# Autodesk Inventor assembly: Eje z base
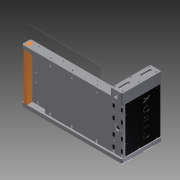
[picture p0: Inventor's stored thumbnail of the model, 180x180]
Saved by Autodesk Inventor 2012 SP1 (Build 160190100, 190)
## iProperties
Created: 2014-12-27
Part Number: Eje z base
Document SubType Name: Assembly
Designer: PRINCIPAL
Author: PRINCIPAL
## Documents named in this file (13)
- E:\impresora juan marc albert\Ultima modificacio Impresora\modificacio chasis 1-9-14\eje z nuevo\Eje z base.iam
- E:\impresora juan marc albert\Ultima modificacio Impresora\modificacio chasis 1-9-14\eje z nuevo\brazo eje z.ipt
- E:\impresora juan marc albert\cojinete lm10uu.ipt
- E:\impresora juan marc albert\Ultima modificacio Impresora\modificacio chasis 1-9-14\eje z nuevo\pieza central base superior.ipt
- E:\impresora juan marc albert\Ultima modificacio Impresora\modificacio chasis 1-9-14\eje z nuevo\pieza central base inferior.ipt
- E:\impresora juan marc albert\Ultima modificacio Impresora\modificacio chasis 1-9-14\eje z nuevo\frontal mes nom.ipt
- E:\impresora juan marc albert\Ultima modificacio Impresora\modificacio chasis 1-9-14\eje z nuevo\base.ipt
- E:\impresora juan marc albert\Ultima modificacio Impresora\modificacio chasis 1-9-14\eje z nuevo\IMAN + ESFERA 6.ipt
- E:\impresora juan marc albert\Ultima modificacio Impresora\modificacio chasis 1-9-14\eje z nuevo\suport iman.ipt
- E:\impresora juan marc albert\Ultima modificacio Impresora\modificacio chasis 1-9-14\eje z nuevo\suport z darrera.ipt
- E:\impresora juan marc albert\Ultima modificacio Impresora\modificacio chasis 1-9-14\eje z nuevo\frontal base reforç.ipt
- E:\impresora juan marc albert\Ultima modificacio Impresora\modificacio chasis 1-9-14\eje z nuevo\suplemento cojinete.ipt
- E:\impresora juan marc albert\Ultima modificacio Impresora\modificacio chasis 1-9-14\eje z nuevo\suplemento cojinete tapa.ipt
## Components (22 placed, 12 different names)
1. brazo eje z:1 — Coincidencia:1, Coincidencia:2, Tangente:1, Tangente:2, Tangente:3, Tangente:4, Ángulo:1, Ángulo:2, Nivelación:1, Nivelación:2, Nivelación:5, Coincidencia:6, Nivelación:4, Coincidencia:14
2. brazo eje z:2 — Coincidencia:3, Coincidencia:4, Tangente:5, Tangente:6, Tangente:7, Tangente:8, Tangente:9, Ángulo:1, Ángulo:2, Nivelación:1, Nivelación:2, Nivelación:3, Coincidencia:5, Nivelación:6, Coincidencia:11, Coincidencia:12, Nivelación:10, Coincidencia:17, Insertar:29
3. cojinete lm10uu:1 — Coincidencia:4, Tangente:8, Tangente:9
4. cojinete lm10uu:2 — Coincidencia:3, Tangente:5, Tangente:6, Tangente:7
5. cojinete lm10uu:3 — Coincidencia:2, Tangente:1, Tangente:2
6. cojinete lm10uu:4 — Coincidencia:1, Tangente:3, Tangente:4
7. pieza central base superior:1 — Nivelación:3, Coincidencia:5, Nivelación:4, Nivelación:5, Ángulo:3, Ángulo:5, Ángulo:6, Ángulo:7, Insertar:17, Insertar:18, Insertar:19, Insertar:20, Insertar:21, Insertar:22
8. pieza central base inferior:1 — Coincidencia:6, Nivelación:6, Nivelación:11, Coincidencia:15, Coincidencia:16
9. frontal mes nom:1 — Coincidencia:11, Coincidencia:12, Nivelación:10, Ángulo:4
10. base:1 — Ángulo:3, Ángulo:4, Insertar:26, Insertar:27, Insertar:28
11. IMAN + ESFERA 6:1 — Insertar:25, Insertar:28
12. IMAN + ESFERA 6:2 — Insertar:24, Insertar:26
13. IMAN + ESFERA 6:3 — Insertar:23, Insertar:27
14. suport iman:1 — Ángulo:6, Insertar:17, Insertar:18, Insertar:23
15. suport iman:2 — Ángulo:7, Insertar:19, Insertar:20, Insertar:24
16. suport iman:3 — Ángulo:5, Insertar:21, Insertar:22, Insertar:25
17. suport z darrera:1 — Nivelación:11, Coincidencia:14
18. frontal base reforç:1 — Coincidencia:15, Coincidencia:16, Coincidencia:17
19. suplemento cojinete:1 — Insertar:29, Insertar:30, Insertar:31
20. suplemento cojinete tapa:1 — Insertar:34
21. suplemento cojinete:2 — Insertar:30, Insertar:31, Insertar:32, Insertar:33
22. suplemento cojinete:3 — Insertar:32, Insertar:33, Insertar:34
## Relationships (54: Insert 18, Mate 12, Tangent 9, Flush 8, Angle 7)
- Coincidencia:1 [Mate]: brazo eje z:1 ↔ cojinete lm10uu:4
- Coincidencia:2 [Mate]: brazo eje z:1 ↔ cojinete lm10uu:3
- Coincidencia:3 [Mate]: brazo eje z:2 ↔ cojinete lm10uu:2
- Coincidencia:4 [Mate]: brazo eje z:2 ↔ cojinete lm10uu:1
- Tangente:1: brazo eje z:1 ↔ cojinete lm10uu:3
- Tangente:2: brazo eje z:1 ↔ cojinete lm10uu:3
- Tangente:3: brazo eje z:1 ↔ cojinete lm10uu:4
- Tangente:4: brazo eje z:1 ↔ cojinete lm10uu:4
- Tangente:5: brazo eje z:2 ↔ cojinete lm10uu:2
- Tangente:6: brazo eje z:2 ↔ cojinete lm10uu:2
- Tangente:7: brazo eje z:2 ↔ cojinete lm10uu:2
- Tangente:8: brazo eje z:2 ↔ cojinete lm10uu:1
- Tangente:9: brazo eje z:2 ↔ cojinete lm10uu:1
- Ángulo:1 [Angle] (0 deg): brazo eje z:1 ↔ brazo eje z:2
- Ángulo:2 [Angle] (0 deg): brazo eje z:1 ↔ brazo eje z:2
- Nivelación:1 [Flush]: brazo eje z:1 ↔ brazo eje z:2
- Nivelación:2 [Flush]: brazo eje z:1 ↔ brazo eje z:2
- Nivelación:3 [Flush]: brazo eje z:2 ↔ pieza central base superior:1
- Coincidencia:5 [Mate]: brazo eje z:2 ↔ pieza central base superior:1
- Nivelación:4 [Flush]: brazo eje z:1 ↔ pieza central base superior:1
- Nivelación:5 [Flush]: brazo eje z:1 ↔ pieza central base superior:1
- Coincidencia:6 [Mate]: brazo eje z:1 ↔ pieza central base inferior:1
- Nivelación:6 [Flush]: brazo eje z:2 ↔ pieza central base inferior:1
- Coincidencia:11 [Mate]: brazo eje z:2 ↔ frontal mes nom:1
- Coincidencia:12 [Mate]: brazo eje z:2 ↔ frontal mes nom:1
- Nivelación:10 [Flush]: brazo eje z:2 ↔ frontal mes nom:1
- Ángulo:3 [Angle] (0 deg): pieza central base superior:1 ↔ base:1
- Ángulo:4 [Angle] (0 deg): frontal mes nom:1 ↔ base:1
- Ángulo:5 [Angle] (0 deg): pieza central base superior:1 ↔ suport iman:3
- Ángulo:6 [Angle] (0 deg): pieza central base superior:1 ↔ suport iman:1
- Ángulo:7 [Angle] (0 deg): pieza central base superior:1 ↔ suport iman:2
- Insertar:17: pieza central base superior:1 ↔ suport iman:1
- Insertar:18: pieza central base superior:1 ↔ suport iman:1
- Insertar:19: pieza central base superior:1 ↔ suport iman:2
- Insertar:20: pieza central base superior:1 ↔ suport iman:2
- Insertar:21: pieza central base superior:1 ↔ suport iman:3
- Insertar:22: pieza central base superior:1 ↔ suport iman:3
- Insertar:23: IMAN + ESFERA 6:3 ↔ suport iman:1
- Insertar:24: IMAN + ESFERA 6:2 ↔ suport iman:2
- Insertar:25: IMAN + ESFERA 6:1 ↔ suport iman:3
- Insertar:26: base:1 ↔ IMAN + ESFERA 6:2
- Insertar:27: base:1 ↔ IMAN + ESFERA 6:3
- Insertar:28: base:1 ↔ IMAN + ESFERA 6:1
- Nivelación:11 [Flush]: pieza central base inferior:1 ↔ suport z darrera:1
- Coincidencia:14 [Mate]: brazo eje z:1 ↔ suport z darrera:1
- Coincidencia:15 [Mate]: pieza central base inferior:1 ↔ frontal base reforç:1
- Coincidencia:16 [Mate]: pieza central base inferior:1 ↔ frontal base reforç:1
- Coincidencia:17 [Mate]: brazo eje z:2 ↔ frontal base reforç:1
- Insertar:29: brazo eje z:2 ↔ suplemento cojinete:1
- Insertar:30: suplemento cojinete:1 ↔ suplemento cojinete:2
- Insertar:31: suplemento cojinete:1 ↔ suplemento cojinete:2
- Insertar:32: suplemento cojinete:2 ↔ suplemento cojinete:3
- Insertar:33: suplemento cojinete:2 ↔ suplemento cojinete:3
- Insertar:34: suplemento cojinete tapa:1 ↔ suplemento cojinete:3
